# Autodesk Inventor assembly: FullAssemSDA
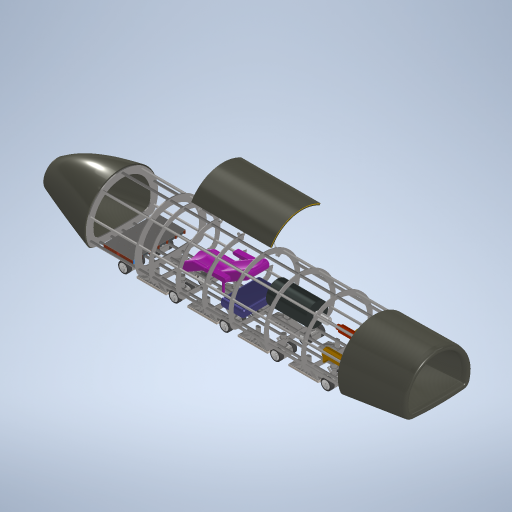
[picture p0: Inventor's stored thumbnail of the model, 512x512]
Saved by Autodesk Inventor 2023 (Build 270158000, 158)
## iProperties
Created: 2022-09-11
Part Number: FullAssemSDA
Document SubType Name: Assembly
Designer: Administrator
Title: FullAssemSDA v3
Author: Administrator
## Documents named in this file (17)
- C:\Users\saver\OneDrive\LongPod\LongPod\FullAssemSDA.iam
- C:\Users\saver\OneDrive\LongPod\LongPod\PodStructure_5.iam
- C:\Users\saver\OneDrive\LongPod\LongPod\tail skin.ipt
- C:\Users\saver\OneDrive\LongPod\LongPod\nose_skin.ipt
- C:\Users\saver\OneDrive\LongPod\LongPod\Air_Bearing_2.2.iam
- C:\Users\saver\OneDrive\LongPod\LongPod\01_dssl_landing_asm_asm.iam
- C:\Users\saver\OneDrive\LongPod\LongPod\DoorSubAssy_5.iam
- C:\Users\saver\OneDrive\LongPod\LongPod\ActuatorRod.ipt
- C:\Users\saver\OneDrive\LongPod\LongPod\LinearActuator.ipt
- C:\Users\saver\OneDrive\LongPod\LongPod\Doorhinge_5.ipt
- C:\Users\saver\OneDrive\LongPod\LongPod\dssl_seatingasm_asm_ScaledDown_0.8.ipt
- C:\Users\saver\OneDrive\LongPod\LongPod\11_7_15 - 60 cell flat Version.iam
- C:\Users\saver\OneDrive\LongPod\LongPod\propeller.ipt
- C:\Users\saver\OneDrive\LongPod\LongPod\JETCATP200.ipt
- C:\Users\saver\OneDrive\LongPod\LongPod\Rough Tesla Rear Motor Model.ipt
- C:\Users\saver\OneDrive\LongPod\LongPod\9827K500_9827K5.ipt
- C:\Users\saver\OneDrive\LongPod\LongPod\Cooling Tank.ipt
## Components (37 placed, 16 different names)
1. PodStructure_5:1 [sub-assembly] — Mate:6, Mate:7, Mate:8, Mate:14
2. tail skin:1
3. nose_skin:1
4. Air_Bearing_2.2:1 [sub-assembly]
5. Air_Bearing_2.2:2 [sub-assembly]
6. Air_Bearing_2.2:3 [sub-assembly]
7. Air_Bearing_2.2:4 [sub-assembly]
8. Air_Bearing_2.2:5 [sub-assembly]
9. Air_Bearing_2.2:6 [sub-assembly]
10. Air_Bearing_2.2:7 [sub-assembly]
11. Air_Bearing_2.2:8 [sub-assembly]
12. 01_dssl_landing_asm_asm:1 [sub-assembly]
13. 01_dssl_landing_asm_asm:2 [sub-assembly]
14. 01_dssl_landing_asm_asm:3 [sub-assembly]
15. 01_dssl_landing_asm_asm:4 [sub-assembly]
16. 01_dssl_landing_asm_asm:5 [sub-assembly]
17. 01_dssl_landing_asm_asm:6 [sub-assembly]
18. 01_dssl_landing_asm_asm:7 [sub-assembly]
19. 01_dssl_landing_asm_asm:8 [sub-assembly]
20. 01_dssl_landing_asm_asm:9 [sub-assembly]
21. 01_dssl_landing_asm_asm:10 [sub-assembly]
22. DoorSubAssy_5:1 [sub-assembly] — Mate:1, Mate:2, Mate:4, Mate:5, Mate:8, Mate:9, Mate:10, Mate:11, Mate:12
23. ActuatorRod:1 — Mate:3, Mate:4, Mate:5
24. ActuatorRod:2 — Mate:11, Mate:12, Mate:13
25. LinearActuator:1 — Mate:13, Mate:14
26. LinearActuator:2 — Mate:3, Mate:6, Mate:7
27. Doorhinge_5:1 — Mate:9, Flush:1, Mate:10
28. Doorhinge_5:2 — Mate:1, Mate:2, Flush:1
29. dssl_seatingasm_asm_ScaledDown_0.8:1
30. 11_7_15 - 60 cell flat Version:1 [sub-assembly]
31. propeller:1
32. JETCATP200:1
33. JETCATP200:2
34. Rough Tesla Rear Motor Model:1
35. 9827K500_9827K5:1
36. 9827K500_9827K5:2
37. Cooling Tank:1
## Relationships (15: Mate 14, Flush 1)
- Mate:1: DoorSubAssy_5:1 ↔ Doorhinge_5:2
- Mate:2: DoorSubAssy_5:1 ↔ Doorhinge_5:2
- Mate:3: ActuatorRod:1 ↔ LinearActuator:2
- Mate:4: DoorSubAssy_5:1 ↔ ActuatorRod:1
- Mate:5: DoorSubAssy_5:1 ↔ ActuatorRod:1
- Mate:6: PodStructure_5:1 ↔ LinearActuator:2
- Mate:7 (6.35 mm): PodStructure_5:1 ↔ LinearActuator:2
- Mate:8: PodStructure_5:1 ↔ DoorSubAssy_5:1
- Mate:9: DoorSubAssy_5:1 ↔ Doorhinge_5:1
- Flush:1: Doorhinge_5:1 ↔ Doorhinge_5:2
- Mate:10: DoorSubAssy_5:1 ↔ Doorhinge_5:1
- Mate:11: DoorSubAssy_5:1 ↔ ActuatorRod:2
- Mate:12: DoorSubAssy_5:1 ↔ ActuatorRod:2
- Mate:13: ActuatorRod:2 ↔ LinearActuator:1
- Mate:14: PodStructure_5:1 ↔ LinearActuator:1
